# Autodesk Inventor assembly: Hotend v6
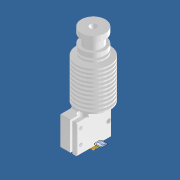
[picture p0: Inventor's stored thumbnail of the model, 180x180]
Saved by Autodesk Inventor 2020 (Build 240168000, 168)
## iProperties
Created: 2021-04-04
Part Number: Hotend v6
Document SubType Name: Assembly
Designer: ken113
Author: ken113
## Documents named in this file (3)
- D:\Document\Github\Cheap_Belt_Printer\Model\Parts\Hotend\hotend-e3d-volcano-1.snapshot.3\Hotend v6.iam
- D:\Document\Github\Cheap_Belt_Printer\Model\Parts\Hotend\hotend-e3d-volcano-1.snapshot.3\V6_VolcanoHotend v6.iam
- D:\Document\Github\Cheap_Belt_Printer\Model\Parts\Hotend\E3D_V6\Nozzel\Sharp_V6_Nozzle.ipt
## Components (2 placed, 2 different names)
1. V6_VolcanoHotend v6:1 [sub-assembly] — リジッド:1
2. Sharp_V6_Nozzle:2 — リジッド:1
## Relationships (1: WeldJoint 1)
- リジッド:1 [WeldJoint]: V6_VolcanoHotend v6:1 ↔ Sharp_V6_Nozzle:2
